# Autodesk Inventor assembly: Diffbox_v2
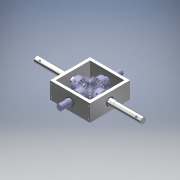
[picture p0: Inventor's stored thumbnail of the model, 180x180]
Saved by Autodesk Inventor 2018 (Build 220112000, 112)
## iProperties
Created: 2017-10-20
Part Number: Diffbox_v2
Material: 一般
Document SubType Name: Assembly
Designer: 翔
Mass: 2050.26 g
Surface Area: 1373.09 cm^2
Volume: 491.149 cm^3
Density: 4.17441 g/cm^3
Author: 翔
## Documents named in this file (7)
- E:\forest_robot_cad\Forest_v4\Diffbox\Diffbox_v2.iam
- E:\forest_robot_cad\Forest_v4\Diffbox\Differential_Gear_Box.iam
- E:\forest_robot_cad\Forest_v4\Diffbox\Shaft_satellite.ipt
- E:\forest_robot_cad\Forest_v4\Diffbox\Diffbox_plate_satelite.ipt
- E:\forest_robot_cad\Forest_v4\bearling\Diffbox_bear_6704DD.ipt
- E:\forest_robot_cad\Forest_v4\Diffbox\Diffbox_plate_main.ipt
- E:\forest_robot_cad\Forest_v4\Diffbox\Shaft_main.ipt
## Components (13 placed, 6 different names)
1. Differential_Gear_Box:1 [sub-assembly] — メイト:1, メイト:2, メイト:3, メイト:4, メイト:5, メイト:23, メイト:24, メイト:25, メイト:26
2. Shaft_satellite:1 — メイト:1, メイト:2, メイト:3, メイト:8, メイト:9
3. Shaft_satellite:2 — メイト:4, メイト:5, メイト:12, メイト:13
4. Diffbox_plate_satelite:1 — メイト:6, メイト:7, メイト:9, フラッシュ:1, メイト:17
5. Diffbox_bear_6704DD:1 — メイト:6, メイト:7, メイト:8
6. Diffbox_plate_satelite:2 — メイト:13, フラッシュ:1, フラッシュ:2, フラッシュ:3, メイト:14, メイト:15, メイト:16
7. Diffbox_bear_6704DD:2 — メイト:12
8. Diffbox_plate_main:1 — フラッシュ:2, メイト:16, メイト:17, メイト:20, メイト:21
9. Diffbox_plate_main:2 — フラッシュ:3, メイト:14, メイト:15, メイト:18, メイト:19
10. Diffbox_bear_6704DD:3 — メイト:18, メイト:19
11. Diffbox_bear_6704DD:4 — メイト:20, メイト:21
12. Shaft_main:1 — メイト:23, メイト:26
13. Shaft_main:2 — メイト:24, メイト:25
## Relationships (28: Mate 25, Flush 3)
- メイト:1 [Mate]: Differential_Gear_Box:1 ↔ Shaft_satellite:1
- メイト:2 [Mate]: Differential_Gear_Box:1 ↔ Shaft_satellite:1
- メイト:3 [Mate]: Differential_Gear_Box:1 ↔ Shaft_satellite:1
- メイト:4 [Mate]: Differential_Gear_Box:1 ↔ Shaft_satellite:2
- メイト:5 [Mate]: Differential_Gear_Box:1 ↔ Shaft_satellite:2
- メイト:6 [Mate]: Diffbox_plate_satelite:1 ↔ Diffbox_bear_6704DD:1
- メイト:7 [Mate]: Diffbox_plate_satelite:1 ↔ Diffbox_bear_6704DD:1
- メイト:8 [Mate]: Shaft_satellite:1 ↔ Diffbox_bear_6704DD:1
- メイト:9 [Mate]: Shaft_satellite:1 ↔ Diffbox_plate_satelite:1
- [Mate]: Diffbox_plate_satelite:2 ↔ Diffbox_bear_6704DD:2
- [Mate]: Diffbox_plate_satelite:2 ↔ Diffbox_bear_6704DD:2
- メイト:12 [Mate]: Shaft_satellite:2 ↔ Diffbox_bear_6704DD:2
- メイト:13 [Mate]: Shaft_satellite:2 ↔ Diffbox_plate_satelite:2
- フラッシュ:1 [Flush]: Diffbox_plate_satelite:1 ↔ Diffbox_plate_satelite:2
- フラッシュ:2 [Flush]: Diffbox_plate_satelite:2 ↔ Diffbox_plate_main:1
- フラッシュ:3 [Flush]: Diffbox_plate_satelite:2 ↔ Diffbox_plate_main:2
- メイト:14 [Mate]: Diffbox_plate_satelite:2 ↔ Diffbox_plate_main:2
- メイト:15 [Mate]: Diffbox_plate_satelite:2 ↔ Diffbox_plate_main:2
- メイト:16 [Mate]: Diffbox_plate_satelite:2 ↔ Diffbox_plate_main:1
- メイト:17 [Mate]: Diffbox_plate_satelite:1 ↔ Diffbox_plate_main:1
- メイト:18 [Mate]: Diffbox_plate_main:2 ↔ Diffbox_bear_6704DD:3
- メイト:19 [Mate]: Diffbox_plate_main:2 ↔ Diffbox_bear_6704DD:3
- メイト:20 [Mate]: Diffbox_plate_main:1 ↔ Diffbox_bear_6704DD:4
- メイト:21 [Mate]: Diffbox_plate_main:1 ↔ Diffbox_bear_6704DD:4
- メイト:23 [Mate]: Differential_Gear_Box:1 ↔ Shaft_main:1
- メイト:24 [Mate]: Differential_Gear_Box:1 ↔ Shaft_main:2
- メイト:25 [Mate]: Differential_Gear_Box:1 ↔ Shaft_main:2
- メイト:26 [Mate]: Differential_Gear_Box:1 ↔ Shaft_main:1
## Named parameters: d9_d5 = 0 mm, d10_d6 = 0 mm
